# Autodesk Inventor assembly: modul_napedowy
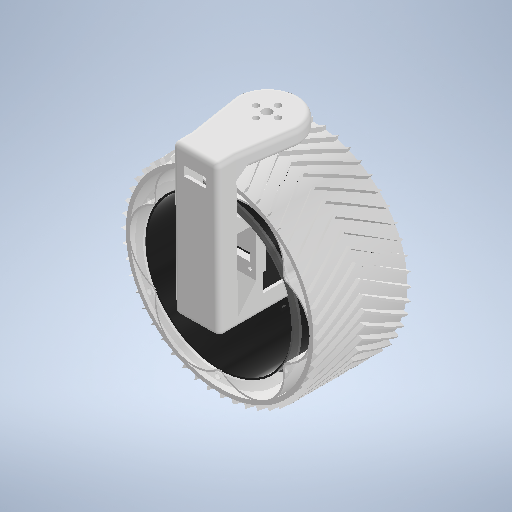
[picture p0: Inventor's stored thumbnail of the model, 512x512]
Saved by Autodesk Inventor 2025.3 (Build 293356000, 356)
## iProperties
Created: 2026-05-07
Part Number: modul_napedowy
Document SubType Name: Assembly
Designer: ksawe
Author: ksawe
## Documents named in this file (4)
- C:\Users\ksawe\OneDrive\Pulpit\Exomy v1\wersja3\modul_napedowy.iam
- C:\Users\ksawe\OneDrive\Pulpit\Exomy v1\wersja3\Kolov2.iam
- C:\Users\ksawe\OneDrive\Pulpit\Exomy v1\wersja3\wahaczv2.ipt
- C:\Users\ksawe\OneDrive\Pulpit\Exomy v1\wersja3\serwo.iam
## Components (3 placed, 3 different names)
1. Kolov2:1 [sub-assembly] — Rigid:2
2. wahaczv2:1 — Rigid:1
3. serwo:1 [sub-assembly] — Rigid:1, Rigid:2
## Relationships (2: WeldJoint 2)
- Rigid:1 [WeldJoint]: wahaczv2:1 ↔ serwo:1
- Rigid:2 [WeldJoint]: Kolov2:1 ↔ serwo:1
